# Autodesk Inventor assembly: Placed cabinet drawer and 2 doors
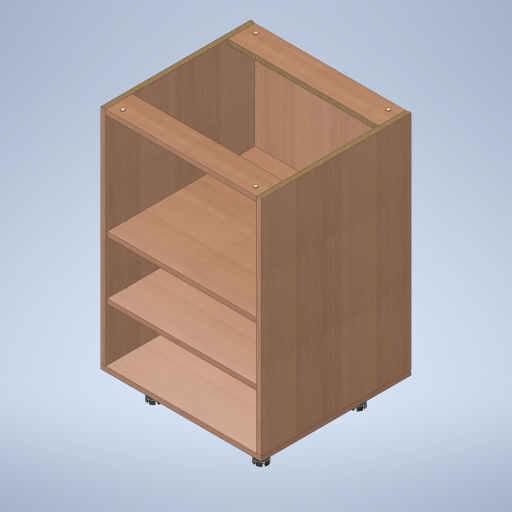
[picture p0: Inventor's stored thumbnail of the model, 512x512]
Saved by Autodesk Inventor 2024 (Build 280153000, 153)
## iProperties
RuleStatus: InUse
Created: 2017-02-06
Part Number: Placed cabinet drawer and 2 doors
Document SubType Name: Assembly
Designer: SvetlanaB
Author: SvetlanaB
## Documents named in this file (20)
- C:\W4INV 2024 Design\iBOX LIBRARY\Kitchen\Standing Cabinets\Cabinet with shelves\Cabinet with shelves.iam
- C:\W4INV 2024 Design\iBOX LIBRARY\Kitchen\Standing Cabinets\Cabinet with shelves\Right panel.ipt
- C:\W4INV 2024 Design\iBOX LIBRARY\Kitchen\Standing Cabinets\Cabinet with shelves\Bottom panel.ipt
- C:\W4INV 2024 Design\iBOX LIBRARY\Kitchen\Standing Cabinets\Cabinet with shelves\Left panel.ipt
- C:\W4INV 2024 Design\iBOX LIBRARY\Kitchen\Standing Cabinets\Cabinet with shelves\Back panel.ipt
- C:\W4INV 2024 Design\iBOX LIBRARY\Kitchen\Standing Cabinets\Cabinet with shelves\Shelf.ipt
- C:\W4INV 2024 Design\iBOX LIBRARY\Kitchen\Standing Cabinets\Cabinet with shelves\Top panel.ipt
- C:\W4INV 2024 Design\iBOX LIBRARY\Kitchen\Standing Cabinets\Cabinet with shelves\Cabinet with shelfs.ipt
- C:\W4INV 2024 Design\_LIBRARY\Holders\Shelf holder D5\Shelf support D5 L16 with hole covers.ipt
- C:\W4INV 2024 Design\_LIBRARY\Supports and legs\Legs\ADJUSTABLE LEG\Adjustable leg  BT18 clip included.ipt
- C:\W4INV 2024 Design\_LIBRARY\Supports and legs\Legs\ADJUSTABLE LEG\Adjustable leg  BT18.ipt
- C:\W4INV 2024 Design\_LIBRARY\Fixed joints\Confirmat\CONFIRMAT\Confirmat L50 NB T18 PB T 18.ipt
- C:\W4INV 2024 Design\_LIBRARY\Fixed joints\Minifix joint\MINIFIX D15 v2\Minifix D15 & Dowel L34 & Cap D15 PB T18 LH.ipt
- C:\W4INV 2024 Design\_LIBRARY\Fixed joints\Minifix joint\MINIFIX D15 v2\Minifix D15 & Dowel L34 & Cap D15 PB T18 RH.ipt
- C:\W4INV 2024 Design\_LIBRARY\Fixed joints\Confirmat\CONFIRMAT\Confirmat L50 & Cap D10 NB T18 PB T 18.ipt
- C:\W4INV 2024 Design\iBOX LIBRARY\Kitchen\Standing Cabinets\Cabinet with shelves\Top panel 2.ipt
- C:\W4INV 2023 Design\LIBRARY\Fixed joints\Confirmat\CONFIRMAT.ipt
- C:\W4INV 2023 Design\LIBRARY\Fixed joints\Minifix joint\MINIFIX D15 v2.ipt
- C:\W4INV 2023 Design\LIBRARY\Holders\Shelf holder D5.ipt
- C:\W4INV 2023 Design\LIBRARY\Supports and legs\Legs\ADJUSTABLE LEG.ipt
## Components (29 placed, 15 different names)
1. @Skeleton
2. Right panel:1 — Side Board Plane:3, Side Board Plane:4, Flush:15, Flush:16, Flush:17, Pillar Board Side Plane:5, Pillar Board Side Plane:7, Nestled Board Plane:1, Nestled Board Plane:4, Mate:77
3. Bottom panel:1 — Bottom board Plane:1, Front (Angle) Plane:1, Bottom board Plane:2, Front (Angle) Plane:2, Bottom board Plane:3, Bottom board Plane:4, Nestled Board Plane:5, Nestled Board Plane:6, Nestled Board Plane:7, Nestled Board Plane:8
4. Left panel:1 — Flush:3, Flush:4, Side Board Plane:1, Side Board Plane:2, Flush:18, Pillar Board Side Plane:6, Pillar Board Side Plane:8, Nestled Board Plane:2, Nestled Board Plane:3, Mate:76, Flush:34
5. Back panel:1 — Mate:76, Flush:34, Mate:77
6. Top panel:1 — Flush:29, Pillar Board Side Plane :2, Pillar Board Side Plane :1
7. Adjustable leg  BT18 clip included:1 — Axis Plane:13, Bottom board Plane:1, Axis2 Plane:1, Front (Angle) Plane:1
8. Adjustable leg  BT18 clip included:2 — Axis Plane:14, Bottom board Plane:2, Axis2 Plane:2, Front (Angle) Plane:2
9. Adjustable leg  BT18:3 — Axis Plane:15, Bottom board Plane:3, Axis2 Plane:3
10. Adjustable leg  BT18:4 — Axis Plane:16, Bottom board Plane:4, Axis2 Plane:4
11. Confirmat L50 & Cap D10 NB T18 PB T 18:5 — Axis Plane:9, Pillar Board Side Plane:5, Nestled Board Plane:5
12. Confirmat L50 NB T18 PB T 18:6 — Axis Plane:10, Pillar Board Side Plane:6, Nestled Board Plane:6
13. Confirmat L50 NB T18 PB T 18:7 — Axis Plane:11, Pillar Board Side Plane:7, Nestled Board Plane:7
14. Confirmat L50 NB T18 PB T 18:8 — Axis Plane:12, Pillar Board Side Plane:8, Nestled Board Plane:8
15. Minifix D15 & Dowel L34 & Cap D15 PB T18 RH:1 — Nestled Board Plane:1, Axis Plane:5, Pillar Board Side Plane :1
16. Minifix D15 & Dowel L34 & Cap D15 PB T18 LH:2 — Nestled Board Plane:2, Axis Plane:6, Pillar Board Side Plane :2
17. Minifix D15 & Dowel L34 & Cap D15 PB T18 RH:3 — Nestled Board Plane:3, Axis Plane:7, Pillar Board Side Plane :3
18. Minifix D15 & Dowel L34 & Cap D15 PB T18 LH:4 — Nestled Board Plane:4, Axis Plane:8, Pillar Board Side Plane :4
19. Top panel 2:1 — Flush:37, Pillar Board Side Plane :4, Pillar Board Side Plane :3
20. Shelf:1 — Shelf Pottom Plane:3, Shelf Pottom Plane:4, Shelf Pottom Plane:1, Shelf Pottom Plane:2
21. Shelf support D5 L16 with hole covers:1 — Axis Plane:1, Side Board Plane:1, Shelf Pottom Plane:1
22. Shelf support D5 L16 with hole covers:2 — Axis Plane:2, Side Board Plane:2, Shelf Pottom Plane:2
23. Shelf support D5 L16 with hole covers:4 — Axis Plane:4, Side Board Plane:4, Shelf Pottom Plane:4
24. Shelf support D5 L16 with hole covers:3 — Axis Plane:3, Side Board Plane:3, Shelf Pottom Plane:3
25. Shelf:2
26. Shelf support D5 L16 with hole covers:5
27. Shelf support D5 L16 with hole covers:6
28. Shelf support D5 L16 with hole covers:7
29. Shelf support D5 L16 with hole covers:8
## Component patterns: (2 elements, first: Shelf:1 + Shelf support D5 L16 with hole covers:1 + Shelf support D5 L16 with hole covers:2 + Shelf support D5 L16 with hole covers:4 + Shelf support D5 L16 with hole covers:3)
## Relationships (61: Mate 42, Flush 17, Angle 2)
- Flush:3 (-64 mm): Left panel:1
- Flush:4 (-64 mm): Left panel:1
- Axis Plane:1 [Mate]: Shelf support D5 L16 with hole covers:1
- Side Board Plane:1 [Mate]: Left panel:1 ↔ Shelf support D5 L16 with hole covers:1
- Axis Plane:2 [Mate]: Shelf support D5 L16 with hole covers:2
- Side Board Plane:2 [Mate]: Left panel:1 ↔ Shelf support D5 L16 with hole covers:2
- Axis Plane:3 [Mate]: Shelf support D5 L16 with hole covers:3
- Side Board Plane:3 [Mate]: Right panel:1 ↔ Shelf support D5 L16 with hole covers:3
- Axis Plane:4 [Mate]: Shelf support D5 L16 with hole covers:4
- Side Board Plane:4 [Mate]: Right panel:1 ↔ Shelf support D5 L16 with hole covers:4
- Flush:15 (-100 mm): Right panel:1
- Flush:16 (-100 mm): Right panel:1
- Flush:17 (-100 mm): Right panel:1
- Flush:18 (-100 mm): Left panel:1
- Axis Plane:13 [Mate]: Adjustable leg  BT18 clip included:1
- Bottom board Plane:1 [Mate]: Bottom panel:1 ↔ Adjustable leg  BT18 clip included:1
- Axis2 Plane:1 [Mate]: Adjustable leg  BT18 clip included:1
- Front (Angle) Plane:1 [Angle] (0 deg): Bottom panel:1 ↔ Adjustable leg  BT18 clip included:1
- Axis Plane:14 [Mate]: Adjustable leg  BT18 clip included:2
- Bottom board Plane:2 [Mate]: Bottom panel:1 ↔ Adjustable leg  BT18 clip included:2
- Axis2 Plane:2 [Mate]: Adjustable leg  BT18 clip included:2
- Front (Angle) Plane:2 [Angle] (0 deg): Bottom panel:1 ↔ Adjustable leg  BT18 clip included:2
- Axis Plane:15 [Mate]: Adjustable leg  BT18:3
- Bottom board Plane:3 [Mate]: Bottom panel:1 ↔ Adjustable leg  BT18:3
- Axis2 Plane:3 [Mate]: Adjustable leg  BT18:3
- Axis Plane:16 [Mate]: Adjustable leg  BT18:4
- Bottom board Plane:4 [Mate]: Bottom panel:1 ↔ Adjustable leg  BT18:4
- Axis2 Plane:4 [Mate]: Adjustable leg  BT18:4
- Axis Plane:9 [Mate]: Confirmat L50 & Cap D10 NB T18 PB T 18:5
- Pillar Board Side Plane:5 [Mate] (-9 mm): Right panel:1 ↔ Confirmat L50 & Cap D10 NB T18 PB T 18:5
- Nestled Board Plane:5 [Flush]: Bottom panel:1 ↔ Confirmat L50 & Cap D10 NB T18 PB T 18:5
- Axis Plane:10 [Mate]: Confirmat L50 NB T18 PB T 18:6
- Pillar Board Side Plane:6 [Mate] (-9 mm): Left panel:1 ↔ Confirmat L50 NB T18 PB T 18:6
- Nestled Board Plane:6 [Flush]: Bottom panel:1 ↔ Confirmat L50 NB T18 PB T 18:6
- Axis Plane:11 [Mate]: Confirmat L50 NB T18 PB T 18:7
- Pillar Board Side Plane:7 [Mate] (-9 mm): Right panel:1 ↔ Confirmat L50 NB T18 PB T 18:7
- Nestled Board Plane:7 [Flush]: Bottom panel:1 ↔ Confirmat L50 NB T18 PB T 18:7
- Axis Plane:12 [Mate]: Confirmat L50 NB T18 PB T 18:8
- Pillar Board Side Plane:8 [Mate] (-9 mm): Left panel:1 ↔ Confirmat L50 NB T18 PB T 18:8
- Nestled Board Plane:8 [Flush]: Bottom panel:1 ↔ Confirmat L50 NB T18 PB T 18:8
- Shelf Pottom Plane:3 [Mate] (2.5 mm): Shelf:1 ↔ Shelf support D5 L16 with hole covers:3
- Shelf Pottom Plane:4 [Mate] (2.5 mm): Shelf:1 ↔ Shelf support D5 L16 with hole covers:4
- Flush:29 (-30 mm): Top panel:1
- Nestled Board Plane:1 [Mate]: Right panel:1 ↔ Minifix D15 & Dowel L34 & Cap D15 PB T18 RH:1
- Axis Plane:5 [Mate]: Minifix D15 & Dowel L34 & Cap D15 PB T18 RH:1
- Nestled Board Plane:2 [Mate]: Left panel:1 ↔ Minifix D15 & Dowel L34 & Cap D15 PB T18 LH:2
- Axis Plane:6 [Mate]: Minifix D15 & Dowel L34 & Cap D15 PB T18 LH:2
- Nestled Board Plane:3 [Mate]: Left panel:1 ↔ Minifix D15 & Dowel L34 & Cap D15 PB T18 RH:3
- Nestled Board Plane:4 [Mate]: Right panel:1 ↔ Minifix D15 & Dowel L34 & Cap D15 PB T18 LH:4
- Shelf Pottom Plane:1 [Mate] (2.5 mm): Shelf:1 ↔ Shelf support D5 L16 with hole covers:1
- Shelf Pottom Plane:2 [Mate] (2.5 mm): Shelf:1 ↔ Shelf support D5 L16 with hole covers:2
- Mate:76: Left panel:1 ↔ Back panel:1
- Flush:34: Left panel:1 ↔ Back panel:1
- Mate:77 (0.5 mm): Right panel:1 ↔ Back panel:1
- Flush:37 (-30 mm): Top panel 2:1
- Axis Plane:8 [Mate]: Minifix D15 & Dowel L34 & Cap D15 PB T18 LH:4
- Axis Plane:7 [Mate]: Minifix D15 & Dowel L34 & Cap D15 PB T18 RH:3
- Pillar Board Side Plane :2 [Flush] (18 mm): Top panel:1 ↔ Minifix D15 & Dowel L34 & Cap D15 PB T18 LH:2
- Pillar Board Side Plane :1 [Flush] (18 mm): Top panel:1 ↔ Minifix D15 & Dowel L34 & Cap D15 PB T18 RH:1
- Pillar Board Side Plane :4 [Flush] (18 mm): Minifix D15 & Dowel L34 & Cap D15 PB T18 LH:4 ↔ Top panel 2:1
- Pillar Board Side Plane :3 [Flush] (18 mm): Minifix D15 & Dowel L34 & Cap D15 PB T18 RH:3 ↔ Top panel 2:1
## Named parameters: Shelf_quantity = 2, Panel_thickness = 18 mm, Top_drawer_place = 180 mm, Distance_between_shelfs = 199.33333 mm
